# Autodesk Inventor assembly: modularRICHFrame
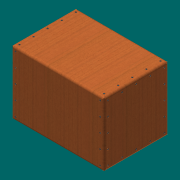
[picture p0: Inventor's stored thumbnail of the model, 180x180]
Saved by Autodesk Inventor 2016 SP1 (Build 200210100, 210)
## iProperties
Created: 2016-04-02
Part Number: modularRICHFrame
Document SubType Name: Assembly
Designer: sawai
Author: sawai
## Documents named in this file (7)
- C:\Users\sawai\OneDrive\projects\modularRICHFrame\modularRICHFrame.iam
- C:\Users\sawai\OneDrive\projects\modularRICHFrame\frame\frame.iam
- C:\Users\sawai\OneDrive\projects\modularRICHFrame\frame\richHolder.iam
- C:\Users\sawai\OneDrive\projects\modularRICHFrame\frame\richHolderSuppourt.iam
- C:\Users\sawai\OneDrive\projects\modularRICHFrame\facing\sideFacing.iam
- C:\Users\sawai\OneDrive\projects\modularRICHFrame\facing\matingORing.ipt
- C:\Users\sawai\OneDrive\projects\modularRICHFrame\facing\frontBackFacing.iam
## Components (12 placed, 6 different names)
1. frame:1 [sub-assembly] — Mate:1, Flush:1, Flush:2, Mate:2, Mate:3, Flush:3, Flush:4, Mate:4, Flush:7, Flush:8, Mate:6, Mate:7, Mate:15, Mate:16
2. richHolder:1 [sub-assembly] — Mate:1, Flush:1, Flush:4, Flush:5, Mate:5
3. richHolder:2 [sub-assembly] — Flush:2, Mate:2, Flush:5, Flush:6
4. richHolderSuppourt:1 [sub-assembly] — Mate:3, Flush:3, Flush:6
5. sideFacing:1 [sub-assembly] — Mate:4, Flush:7, Flush:8, Flush:9, Flush:10, Flush:11, Mate:8, Mate:11, Mate:13, Mate:18, Mate:19
6. sideFacing:2 [sub-assembly] — Mate:5, Flush:9, Mate:10
7. sideFacing:3 [sub-assembly] — Mate:6, Flush:11, Mate:8, Mate:9, Mate:12, Mate:14, Mate:17, Mate:20
8. sideFacing:4 [sub-assembly] — Mate:7, Flush:10, Mate:9, Mate:10
9. matingORing:1 — Mate:11, Mate:12
10. matingORing:2 — Mate:13, Mate:14
11. frontBackFacing:1 [sub-assembly] — Mate:15, Mate:19, Mate:20
12. frontBackFacing:2 [sub-assembly] — Mate:16, Mate:17, Mate:18
## Relationships (31: Mate 20, Flush 11)
- Mate:1: frame:1 ↔ richHolder:1
- Flush:1: frame:1 ↔ richHolder:1
- Flush:2: frame:1 ↔ richHolder:2
- Mate:2: frame:1 ↔ richHolder:2
- Mate:3: frame:1 ↔ richHolderSuppourt:1
- Flush:3: frame:1 ↔ richHolderSuppourt:1
- Flush:4 (-100 mm): frame:1 ↔ richHolder:1
- Flush:5 (-100 mm): richHolder:1 ↔ richHolder:2
- Flush:6 (-100 mm): richHolder:2 ↔ richHolderSuppourt:1
- Mate:4: frame:1 ↔ sideFacing:1
- Flush:7: frame:1 ↔ sideFacing:1
- Flush:8: frame:1 ↔ sideFacing:1
- Mate:5: richHolder:1 ↔ sideFacing:2
- Mate:6: frame:1 ↔ sideFacing:3
- Mate:7: frame:1 ↔ sideFacing:4
- Flush:9: sideFacing:1 ↔ sideFacing:2
- Flush:10: sideFacing:1 ↔ sideFacing:4
- Flush:11: sideFacing:1 ↔ sideFacing:3
- Mate:8: sideFacing:1 ↔ sideFacing:3
- Mate:9: sideFacing:3 ↔ sideFacing:4
- Mate:10: sideFacing:2 ↔ sideFacing:4
- Mate:11: sideFacing:1 ↔ matingORing:1
- Mate:12: sideFacing:3 ↔ matingORing:1
- Mate:13: sideFacing:1 ↔ matingORing:2
- Mate:14: sideFacing:3 ↔ matingORing:2
- Mate:15: frame:1 ↔ frontBackFacing:1
- Mate:16: frame:1 ↔ frontBackFacing:2
- Mate:17: sideFacing:3 ↔ frontBackFacing:2
- Mate:18: sideFacing:1 ↔ frontBackFacing:2
- Mate:19: sideFacing:1 ↔ frontBackFacing:1
- Mate:20: sideFacing:3 ↔ frontBackFacing:1
